# Autodesk Inventor assembly: ThumbProximalPhalanx
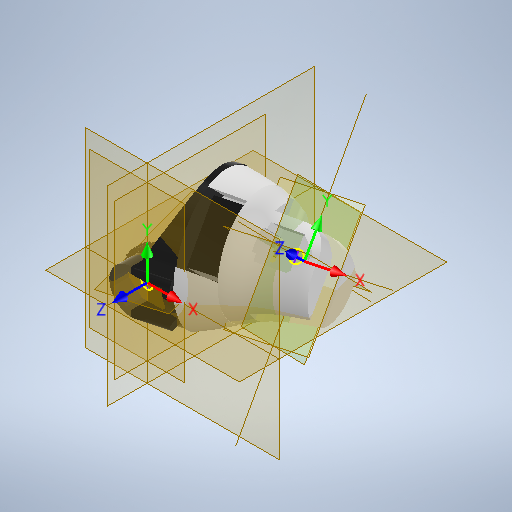
[picture p0: Inventor's stored thumbnail of the model, 512x512]
Saved by Autodesk Inventor 2025.1 (Build 291241000, 241)
## iProperties
Created: 2025-06-06
Part Number: ThumbProximalPhalanx
Document SubType Name: Assembly
Designer: Alexander
Author: Alexander
## Documents named in this file (5)
- D:\Repositorios_Politecnica\Handi-EPN\CAD\Sim Models\ThumbProximalPhalanx.iam
- D:\Repositorios_Politecnica\Handi-EPN\CAD\thumb\MC - D R.ipt
- D:\Repositorios_Politecnica\Handi-EPN\CAD\thumb\MC - P Main R.ipt
- D:\Repositorios_Politecnica\Handi-EPN\CAD\thumb\MC - P Geared Rotator R.ipt
- D:\Repositorios_Politecnica\Handi-EPN\CAD\purchased components (motors, magnets, screws, electronics)\servoMotor\ServoMotor_CaseTH_Interno.iam
## Components (4 placed, 4 different names)
1. MC - D R:1 — Mate:1, Flush:1, Mate:2, Mate:12, Mate:13, Mate:14, Mate:15, Mate:16, Mate:17, Mate:18
2. MC - P Main R:1 — Mate:1, Flush:1, Mate:2, Mate:3, Mate:4, Angle:1, Mate:19, Mate:20
3. MC - P Geared Rotator R:1 — Mate:3, Mate:4, Angle:1, Flush:2, Flush:3, Flush:4, Mate:5
4. ServoMotor_CaseTH_Interno:1 [sub-assembly] — Mate:18, Mate:19, Mate:20
## Relationships (25: Mate 20, Flush 4, Angle 1)
- Mate:1: MC - D R:1 ↔ MC - P Main R:1
- Flush:1 (1.824 mm): MC - D R:1 ↔ MC - P Main R:1
- Mate:2 (17.315 mm): MC - D R:1 ↔ MC - P Main R:1
- Mate:3: MC - P Main R:1 ↔ MC - P Geared Rotator R:1
- Mate:4: MC - P Main R:1 ↔ MC - P Geared Rotator R:1
- Angle:1 (2 deg): MC - P Main R:1 ↔ MC - P Geared Rotator R:1
- Flush:2: MC - P Geared Rotator R:1
- Flush:3: MC - P Geared Rotator R:1
- Flush:4: MC - P Geared Rotator R:1
- Mate:5: MC - P Geared Rotator R:1
- Mate:6
- Mate:7
- Mate:8
- Mate:9
- Mate:10
- Mate:11
- Mate:12: MC - D R:1
- Mate:13: MC - D R:1
- Mate:14: MC - D R:1
- Mate:15: MC - D R:1
- Mate:16: MC - D R:1
- Mate:17: MC - D R:1
- Mate:18: MC - D R:1 ↔ ServoMotor_CaseTH_Interno:1
- Mate:19: MC - P Main R:1 ↔ ServoMotor_CaseTH_Interno:1
- Mate:20: MC - P Main R:1 ↔ ServoMotor_CaseTH_Interno:1
